# Autodesk Inventor assembly: ArmMotorSubAssembly
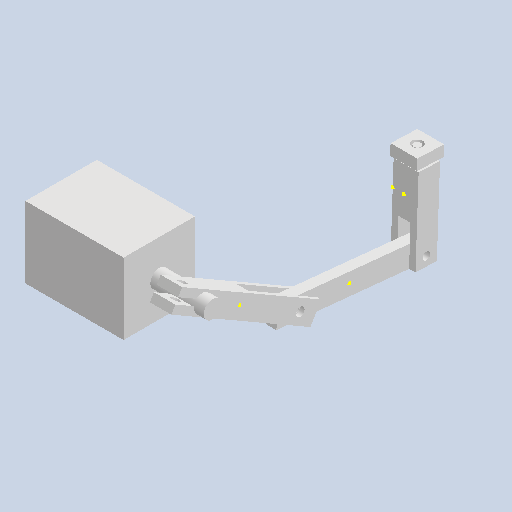
[picture p0: Inventor's stored thumbnail of the model, 512x512]
Saved by Autodesk Inventor 2024 (Build 280153000, 153)
## iProperties
Created: 2023-12-18
Part Number: ArmMotorSubAssembly
Document SubType Name: Assembly
Designer: pratikhya
Author: pratikhya
## Documents named in this file (3)
- C:\Users\prati\OneDrive - IIT Kanpur\Desktop\Robot\ArmMotorSubAssembly.iam
- C:\Users\prati\OneDrive - IIT Kanpur\Desktop\Robot\ArmMotor.ipt
- C:\Users\prati\OneDrive - IIT Kanpur\Desktop\Robot\ArmScaled.ipt
## Components (2 placed, 2 different names)
1. ArmMotor:1 — Rotational:1
2. ArmScaled:1 — Rotational:1
## Relationships (1: RevoluteJoint 1)
- Rotational:1 [RevoluteJoint] (-17.78 mm): ArmMotor:1 ↔ ArmScaled:1
